# Autodesk Inventor assembly: Unterdruckventil
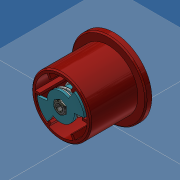
[picture p0: Inventor's stored thumbnail of the model, 180x180]
Saved by Autodesk Inventor 2019 (Build 230136000, 136)
## iProperties
Created: 2020-09-01
Part Number: Unterdruckventil
Material: Generisch
Document SubType Name: Assembly
Designer: Stefan
Mass: 64.2247 g
Surface Area: 301.994 cm^2
Volume: 45.3863 cm^3
Density: 1.41507 g/cm^3
Author: Stefan
## Documents named in this file (7)
- C:\Users\User\OneDrive\Dokumente\Inventor\Absauganlage\Unterdruckventil.iam
- C:\Users\User\OneDrive\Dokumente\Inventor\Absauganlage\Unterdruckventil_Basis.ipt
- C:\Users\User\OneDrive\Dokumente\Inventor\Absauganlage\Unterdruckventil_Membran.ipt
- C:\Users\User\OneDrive\Dokumente\Inventor\Absauganlage\O-Ring_34x3.5.ipt
- C:\Users\User\OneDrive\Dokumente\Inventor\Absauganlage\Unterdruckventil_Gegenhalter.ipt
- C:\Users\User\OneDrive\Dokumente\Inventor\Absauganlage\Unterdruckventil\Konstruktions-Assistent\Druckfeder1.iam
- C:\Users\User\OneDrive\Dokumente\Inventor\Absauganlage\Unterdruckventil\Konstruktions-Assistent\Schraubenverbindung3.iam
## Components (6 placed, 6 different names)
1. Unterdruckventil_Basis:1 — Passend:1, Tangential:2, Passend:3, Passend:12, Passend:13
2. Unterdruckventil_Membran:1 — Passend:1, Passend:2, Tangential:1
3. O-Ring_34x3.5:1 — Passend:2, Tangential:1, Tangential:2
4. Unterdruckventil_Gegenhalter:1 — Passend:3, Passend:7, Fluchtend:1, Passend:11, Passend:14
5. Druckfeder:1 [sub-assembly] — Passend:7, Fluchtend:1
6. Schraubenverbindung:1 [sub-assembly] — Passend:11, Passend:12, Passend:13, Passend:14
## Relationships (11: Mate 8, Tangent 2, Flush 1)
- Passend:1 [Mate]: Unterdruckventil_Basis:1 ↔ Unterdruckventil_Membran:1
- Passend:2 [Mate]: Unterdruckventil_Membran:1 ↔ O-Ring_34x3.5:1
- Tangential:1: Unterdruckventil_Membran:1 ↔ O-Ring_34x3.5:1
- Tangential:2: Unterdruckventil_Basis:1 ↔ O-Ring_34x3.5:1
- Passend:3 [Mate]: Unterdruckventil_Basis:1 ↔ Unterdruckventil_Gegenhalter:1
- Passend:7 [Mate]: Unterdruckventil_Gegenhalter:1 ↔ Druckfeder:1
- Fluchtend:1 [Flush]: Unterdruckventil_Gegenhalter:1 ↔ Druckfeder:1
- Passend:11 [Mate]: Unterdruckventil_Gegenhalter:1 ↔ Schraubenverbindung:1
- Passend:12 [Mate]: Unterdruckventil_Basis:1 ↔ Schraubenverbindung:1
- Passend:13 [Mate]: Unterdruckventil_Basis:1 ↔ Schraubenverbindung:1
- Passend:14 [Mate]: Unterdruckventil_Gegenhalter:1 ↔ Schraubenverbindung:1
